# Autodesk Inventor assembly: Small octopus
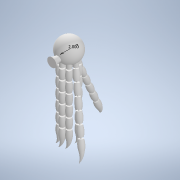
[picture p0: Inventor's stored thumbnail of the model, 180x180]
Saved by Autodesk Inventor 2021 (Build 250183000, 183)
## iProperties
Created: 2020-07-13
Part Number: Small octopus
Document SubType Name: Assembly
Designer: saipr
Author: saipr
## Documents named in this file (3)
- C:\Users\saipr\Desktop\Autodesk 2021\Builds\Parts\Samller Octopus\Small octopus.iam
- C:\Users\saipr\Desktop\Autodesk 2021\Builds\Parts\Samller Octopus\Head.ipt
- C:\Users\saipr\Desktop\Autodesk 2021\Builds\Parts\Samller Octopus\Full Small Tentacle.iam
## Components (9 placed, 2 different names)
1. Head:1 — Mate:1, Mate:2, Mate:3, Mate:4, Mate:5, Mate:6, Mate:7, Mate:8
2. Full Small Tentacle:1 [sub-assembly] — Mate:2
3. Full Small Tentacle:2 [sub-assembly] — Mate:4
4. Full Small Tentacle:3 [sub-assembly] — Mate:5
5. Full Small Tentacle:4 [sub-assembly] — Mate:6
6. Full Small Tentacle:5 [sub-assembly] — Mate:8
7. Full Small Tentacle:6 [sub-assembly] — Mate:1
8. Full Small Tentacle:7 [sub-assembly] — Mate:3
9. Full Small Tentacle:8 [sub-assembly] — Mate:7
## Relationships (8: Mate 8)
- Mate:1: Head:1 ↔ Full Small Tentacle:6
- Mate:2: Head:1 ↔ Full Small Tentacle:1
- Mate:3: Head:1 ↔ Full Small Tentacle:7
- Mate:4: Head:1 ↔ Full Small Tentacle:2
- Mate:5: Head:1 ↔ Full Small Tentacle:3
- Mate:6: Head:1 ↔ Full Small Tentacle:4
- Mate:7: Head:1 ↔ Full Small Tentacle:8
- Mate:8: Head:1 ↔ Full Small Tentacle:5
